# Autodesk Inventor assembly: PH42-020-S300-R
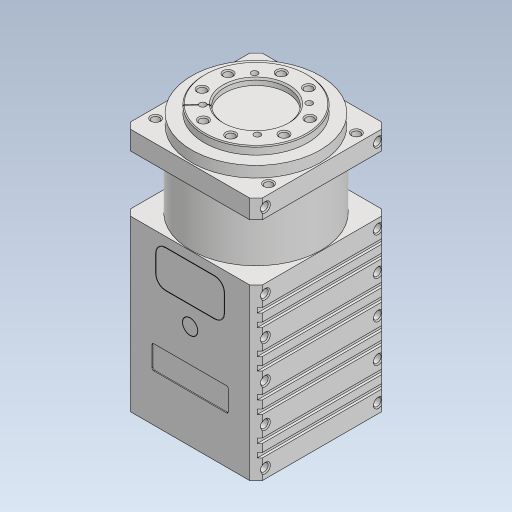
[picture p0: Inventor's stored thumbnail of the model, 512x512]
Saved by Autodesk Inventor 2023 (Build 270158000, 158)
## iProperties
Created: 2023-04-15
Part Number: PH42-020-S300-R
Document SubType Name: Assembly
Designer: michi
Author: michi
## Documents named in this file (3)
- C:\Users\michi\OneDrive - Kyoto University\lab\6_SHINOBI\FUHGA4\Design_Mechanism\Dynamixel\PH42-020\PH42-020-S300-R.iam
- C:\Users\michi\OneDrive - Kyoto University\lab\6_SHINOBI\FUHGA4\Design_Mechanism\Dynamixel\PH42-020\PH42-020-S300-R_body.ipt
- C:\Users\michi\OneDrive - Kyoto University\lab\6_SHINOBI\FUHGA4\Design_Mechanism\Dynamixel\PH42-020\PH42-020-S300-R_hone.ipt
## Components (2 placed, 2 different names)
1. PH42-020-S300-R_body:1 — 挿入:1
2. PH42-020-S300-R_hone:1 — 挿入:1
## Relationships (1: Insert 1)
- 挿入:1 [Insert]: PH42-020-S300-R_body:1 ↔ PH42-020-S300-R_hone:1
